# Autodesk Inventor assembly: ELEV_000_FULLASMBLY
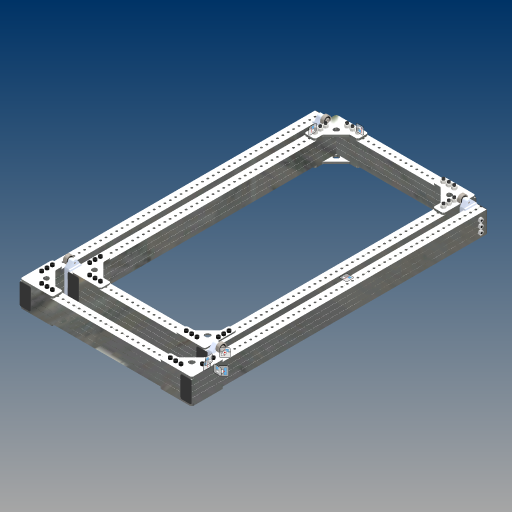
[picture p0: Inventor's stored thumbnail of the model, 512x512]
Saved by Autodesk Inventor 2024.3 (Build 283343000, 343)
## iProperties
Created: 2024-11-25
Part Number: ELEV_000_FULLASMBLY
Document SubType Name: Assembly
Designer: Kenji
Mass: 3407.89 g
Surface Area: 12378 cm^2
Volume: 1206.36 cm^3
Density: 2.82493 g/cm^3
Author: Kenji
## Documents named in this file (25)
- C:\Users\Kenji\Documents\GitHub\1622-2024-Casino-Clash-CAD-A-Thon\Elevator\ELEV_000_FULLASMBLY.iam
- C:\Users\Kenji\Documents\GitHub\1622-2024-Casino-Clash-CAD-A-Thon\Elevator\ELEV_001_BAR1(27.500 in).ipt
- C:\Users\Kenji\Documents\GitHub\1622-2024-Casino-Clash-CAD-A-Thon\Elevator\ELEV_002_BAR2(14.000 in).ipt
- C:\Users\Kenji\Documents\GitHub\1622-2024-Casino-Clash-CAD-A-Thon\Elevator\ELEV_003_BAR3(25.000 in).ipt
- C:\Users\Kenji\Documents\GitHub\1622-2024-Casino-Clash-CAD-A-Thon\COTS Library\Motion\BearingBlocks\ElevatorBlocks\WCP-0897_InlineBearingBlock.iam
- C:\Users\Kenji\Documents\GitHub\1622-2024-Casino-Clash-CAD-A-Thon\Elevator\ELEV_004_BAR4(12.000 in).ipt
- C:\Users\Kenji\Documents\GitHub\1622-2024-Casino-Clash-CAD-A-Thon\Elevator\ELEV_005_SUPBRK1.ipt
- C:\Users\Kenji\Documents\GitHub\1622-2024-Casino-Clash-CAD-A-Thon\COTS Library\Fasteners\Nuts\COTS_90633A411_Low-Strength Steel Thin Nylon-Insert Locknut_10-32.ipt
- C:\Users\Kenji\Documents\GitHub\1622-2024-Casino-Clash-CAD-A-Thon\Elevator\ELEV_006_SUPBRK1_THRD.ipt
- C:\Users\Kenji\Documents\GitHub\1622-2024-Casino-Clash-CAD-A-Thon\COTS Library\Fasteners\Bolts\Socket-Head\10-32\COTS_90044A121_Black-Oxide Alloy Steel Socket Head Screw_10-32_2.5in.ipt
- C:\Users\Kenji\Documents\GitHub\1622-2024-Casino-Clash-CAD-A-Thon\COTS Library\Fasteners\Bolts\Socket-Head\10-32\COTS_90044A202_Black-Oxide Alloy Steel Socket Head Screw_1-.375.ipt
- C:\Users\Kenji\Documents\GitHub\1622-2024-Casino-Clash-CAD-A-Thon\COTS Library\Fasteners\Bolts\Socket-Head\10-32\COTS_91251A342_Black-Oxide Alloy Steel Socket Head Screw_.5in.ipt
- C:\Users\Kenji\Documents\GitHub\1622-2024-Casino-Clash-CAD-A-Thon\Elevator\ELEV_007_SUPBRK2.ipt
- C:\Users\Kenji\Documents\GitHub\1622-2024-Casino-Clash-CAD-A-Thon\COTS Library\Fasteners\Bolts\Socket-Head\10-32\COTS_91251A359_Black-Oxide Alloy Steel Socket Head Screw_10-32_2_3-4in.ipt
- C:\Users\Kenji\Documents\GitHub\1622-2024-Casino-Clash-CAD-A-Thon\COTS Library\Fasteners\Nuts\COTS_90631A411_Low-Strength Steel Nylon-Insert Locknut_10-32.ipt
- C:\Users\Kenji\Documents\GitHub\1622-2024-Casino-Clash-CAD-A-Thon\Elevator\ELEV_008_SUPBRK3.ipt
- C:\Users\Kenji\Documents\GitHub\1622-2024-Casino-Clash-CAD-A-Thon\Elevator\ELEV_009_BOLTCOVER.ipt
- C:\Users\Kenji\Documents\GitHub\1622-2024-Casino-Clash-CAD-A-Thon\Elevator\ELEV_010_BOLTCOVER2.ipt
- C:\Users\Kenji\Documents\GitHub\1622-2024-Casino-Clash-CAD-A-Thon\Elevator\ELEV_011_EXTRUENDCAP.ipt
- C:\Users\Kenji\Documents\GitHub\1622-2024-Casino-Clash-CAD-A-Thon\Elevator\ELEV_000_FULLASMBLY\AIP\FEA\ew6g7bhkw.fins
- C:\Users\Kenji\Documents\GitHub\1622-2024-Casino-Clash-CAD-A-Thon\Elevator\ELEV_000_FULLASMBLY\AIP\FEA\ew6g7bhkw.fsat
- C:\Users\Kenji\Documents\GitHub\1622-2024-Casino-Clash-CAD-A-Thon\Elevator\ELEV_000_FULLASMBLY\AIP\FEA\ew6g7bhkw.ftes
- C:\Users\Kenji\Documents\GitHub\1622-2024-Casino-Clash-CAD-A-Thon\Elevator\ELEV_000_FULLASMBLY\AIP\FEA\ew6g7bhkw.fwiz
- C:\Users\Kenji\Documents\GitHub\1622-2024-Casino-Clash-CAD-A-Thon\Elevator\ELEV_000_FULLASMBLY\AIP\FEA\ew6g7biao.fmsh
- C:\Users\Kenji\Documents\GitHub\1622-2024-Casino-Clash-CAD-A-Thon\Elevator\ELEV_000_FULLASMBLY\AIP\FEA\ew6g7bibk.fres
## Components (151 placed, 18 different names)
1. ELEV_001_BAR1(27.500 in):1 — Flush:1, Flush:2, Mate:1, Mate:2, Flush:7, Tangent:2, Mate:10, Flush:11, Mate:11, Mate:78, Mate:133, Mate:136, Mate:137, Mate:181, Mate:183, Mate:184, Mate:201, Mate:202, Mate:203
2. ELEV_001_BAR1(27.500 in):2 — Flush:1, Flush:2, Mate:1, Flush:3, Flush:4, Mate:3, Angle:1, Mate:4, Flush:8, Angle:2, Mate:74, Mate:128, Mate:131, Mate:178, Mate:180, Mate:182, Mate:198, Mate:199, Mate:200
3. ELEV_002_BAR2(14.000 in):1 — Flush:3, Flush:4, Mate:2, Mate:127, Flush:24, Mate:132, Mate:134, Mate:135
4. ELEV_003_BAR3(25.000 in):1 — Flush:5, Flush:6, Flush:7, Mate:8, Flush:10, Mate:9, Mate:82, Flush:19, Flush:21, Mate:186, Mate:187, Mate:188, Mate:195, Mate:196, Mate:197
5. ELEV_003_BAR3(25.000 in):2 — Flush:5, Flush:6, Tangent:1, Angle:2, Mate:5, Angle:3, Mate:6, Flush:9, Mate:12, Flush:12, Flush:13, Mate:13, Flush:14, Mate:14, Mate:16, Mate:62, Mate:86, Flush:17, Flush:22, Mate:189, Mate:190, Mate:191, Mate:192, Mate:193, Mate:194
6. WCP-0897_InlineBearingBlock:1 [sub-assembly] — Mate:5, Angle:3, Mate:6, Flush:9, Mate:83, Mate:84
7. WCP-0897_InlineBearingBlock:2 [sub-assembly] — Mate:3, Angle:1, Mate:4, Tangent:1, Flush:8, Mate:71, Mate:72
8. WCP-0897_InlineBearingBlock:3 [sub-assembly] — Mate:8, Flush:10, Mate:9, Tangent:2, Mate:79, Mate:80
9. WCP-0897_InlineBearingBlock:4 [sub-assembly] — Mate:10, Flush:11, Mate:11, Mate:75, Mate:76
10. ELEV_004_BAR4(12.000 in):1 — Mate:12, Flush:12, Flush:13, Mate:17, Mate:18, Mate:19, Angle:4, Mate:20, Mate:42, Mate:45, Mate:60, Flush:15, Mate:61
11. ELEV_004_BAR4(12.000 in):2 — Mate:13, Flush:14, Mate:14, Flush:16, Flush:18, Mate:88, Flush:20, Mate:89, Flush:23, Mate:90, Mate:110
12. ELEV_005_SUPBRK1:1 — Mate:16, Mate:17, Mate:18, Mate:67, Mate:68, Mate:69, Mate:70
13. ELEV_005_SUPBRK1:2 — Mate:19, Angle:4, Mate:20, Mate:63, Mate:64, Mate:65, Mate:66
14. ELEV_006_SUPBRK1_THRD:1 — Mate:42, Mate:61, Mate:62, Mate:159, Mate:161
15. ELEV_006_SUPBRK1_THRD:2 — Mate:45, Mate:60, Flush:15, Mate:155, Mate:157
16. ELEV_007_SUPBRK2:1 — Flush:16, Flush:17, Mate:110, Mate:120, Mate:122
17. ELEV_007_SUPBRK2:2 — Flush:18, Flush:19, Mate:88, Mate:124, Mate:126
18. ELEV_007_SUPBRK2:3 — Flush:22, Flush:23, Mate:90, Mate:115, Mate:116, Mate:117, Mate:118
19. ELEV_007_SUPBRK2:4 — Flush:20, Flush:21, Mate:89, Mate:111, Mate:112, Mate:113, Mate:114
20. ELEV_008_SUPBRK3:1 — Mate:127, Flush:24, Mate:128, Mate:129, Mate:130, Mate:138, Mate:139, Mate:144, Mate:145
21. ELEV_008_SUPBRK3:2 — Mate:129, Mate:130, Mate:131, Mate:148, Mate:149
22. ELEV_008_SUPBRK3:3 — Mate:132, Mate:133, Mate:134, Mate:151, Mate:153
23. ELEV_008_SUPBRK3:4 — Mate:135, Mate:136, Mate:137, Mate:140, Mate:141, Mate:142, Mate:143
24. ELEV_011_EXTRUENDCAP:1 — Mate:189, Mate:190, Mate:191
25. ELEV_011_EXTRUENDCAP:2 — Mate:178, Mate:180, Mate:182
26. ELEV_011_EXTRUENDCAP:3 — Mate:186, Mate:187, Mate:188
27. ELEV_011_EXTRUENDCAP:4 — Mate:181, Mate:183, Mate:184
28. ELEV_011_EXTRUENDCAP:5 — Mate:198, Mate:199, Mate:200
29. ELEV_011_EXTRUENDCAP:6 — Mate:201, Mate:202, Mate:203
30. ELEV_011_EXTRUENDCAP:7 — Mate:192, Mate:193, Mate:194
31. ELEV_011_EXTRUENDCAP:8 — Mate:195, Mate:196, Mate:197
32. COTS_90044A121_Black-Oxide Alloy Steel Socket Head Screw_10-32_2.5in:1 — Mate:63, Mate:64
33. COTS_90044A121_Black-Oxide Alloy Steel Socket Head Screw_10-32_2.5in:5
34. COTS_90044A121_Black-Oxide Alloy Steel Socket Head Screw_10-32_2.5in:6 — Mate:156
35. COTS_90044A121_Black-Oxide Alloy Steel Socket Head Screw_10-32_2.5in:4 — Mate:65, Mate:66
36. COTS_90044A121_Black-Oxide Alloy Steel Socket Head Screw_10-32_2.5in:7
37. COTS_90044A121_Black-Oxide Alloy Steel Socket Head Screw_10-32_2.5in:8 — Mate:154
38. COTS_90044A121_Black-Oxide Alloy Steel Socket Head Screw_10-32_2.5in:3 — Mate:68, Mate:70
39. COTS_90044A121_Black-Oxide Alloy Steel Socket Head Screw_10-32_2.5in:9
40. COTS_90044A121_Black-Oxide Alloy Steel Socket Head Screw_10-32_2.5in:10 — Mate:160
41. COTS_90044A121_Black-Oxide Alloy Steel Socket Head Screw_10-32_2.5in:2 — Mate:67, Mate:69
42. COTS_90044A121_Black-Oxide Alloy Steel Socket Head Screw_10-32_2.5in:11
43. COTS_90044A121_Black-Oxide Alloy Steel Socket Head Screw_10-32_2.5in:12 — Mate:158
44. COTS_90044A202_Black-Oxide Alloy Steel Socket Head Screw_1-.375:1 — Mate:71, Mate:72, Mate:73
45. COTS_90633A411_Low-Strength Steel Thin Nylon-Insert Locknut_10-32:1 — Mate:73, Mate:74
46. COTS_90044A202_Black-Oxide Alloy Steel Socket Head Screw_1-.375:2
47. COTS_90633A411_Low-Strength Steel Thin Nylon-Insert Locknut_10-32:2
48. COTS_90044A202_Black-Oxide Alloy Steel Socket Head Screw_1-.375:3
49. COTS_90633A411_Low-Strength Steel Thin Nylon-Insert Locknut_10-32:3
50. COTS_90633A411_Low-Strength Steel Thin Nylon-Insert Locknut_10-32:4 — Mate:77, Mate:78
51. COTS_90044A202_Black-Oxide Alloy Steel Socket Head Screw_1-.375:4 — Mate:75, Mate:76, Mate:77
52. COTS_90633A411_Low-Strength Steel Thin Nylon-Insert Locknut_10-32:5
53. COTS_90044A202_Black-Oxide Alloy Steel Socket Head Screw_1-.375:5
54. COTS_90633A411_Low-Strength Steel Thin Nylon-Insert Locknut_10-32:6
55. COTS_90044A202_Black-Oxide Alloy Steel Socket Head Screw_1-.375:6
56. COTS_91251A342_Black-Oxide Alloy Steel Socket Head Screw_.5in:1 — Mate:79, Mate:80, Mate:81
57. COTS_90633A411_Low-Strength Steel Thin Nylon-Insert Locknut_10-32:7 — Mate:81, Mate:82
58. COTS_91251A342_Black-Oxide Alloy Steel Socket Head Screw_.5in:2
59. COTS_90633A411_Low-Strength Steel Thin Nylon-Insert Locknut_10-32:8
60. COTS_91251A342_Black-Oxide Alloy Steel Socket Head Screw_.5in:3
61. COTS_90633A411_Low-Strength Steel Thin Nylon-Insert Locknut_10-32:9
62. COTS_90633A411_Low-Strength Steel Thin Nylon-Insert Locknut_10-32:10 — Mate:85, Mate:86
63. COTS_91251A342_Black-Oxide Alloy Steel Socket Head Screw_.5in:4 — Mate:83, Mate:84, Mate:85
64. COTS_90633A411_Low-Strength Steel Thin Nylon-Insert Locknut_10-32:11
65. COTS_91251A342_Black-Oxide Alloy Steel Socket Head Screw_.5in:5
66. COTS_90633A411_Low-Strength Steel Thin Nylon-Insert Locknut_10-32:12
67. COTS_91251A342_Black-Oxide Alloy Steel Socket Head Screw_.5in:6
68. COTS_91251A359_Black-Oxide Alloy Steel Socket Head Screw_10-32_2_3-4in:3 — Mate:111, Mate:112, Mate:123, Mate:166
69. COTS_90631A411_Low-Strength Steel Nylon-Insert Locknut_10-32:2 — Mate:123, Mate:124, Mate:168
70. COTS_91251A359_Black-Oxide Alloy Steel Socket Head Screw_10-32_2_3-4in:5
71. COTS_90631A411_Low-Strength Steel Nylon-Insert Locknut_10-32:5
72. COTS_91251A359_Black-Oxide Alloy Steel Socket Head Screw_10-32_2_3-4in:6
73. COTS_90631A411_Low-Strength Steel Nylon-Insert Locknut_10-32:6
74. COTS_91251A359_Black-Oxide Alloy Steel Socket Head Screw_10-32_2_3-4in:1 — Mate:113, Mate:114, Mate:125, Mate:167
75. COTS_91251A359_Black-Oxide Alloy Steel Socket Head Screw_10-32_2_3-4in:7
76. COTS_91251A359_Black-Oxide Alloy Steel Socket Head Screw_10-32_2_3-4in:8
77. COTS_91251A359_Black-Oxide Alloy Steel Socket Head Screw_10-32_2_3-4in:2 — Mate:115, Mate:118, Mate:121, Mate:163
78. COTS_90631A411_Low-Strength Steel Nylon-Insert Locknut_10-32:4 — Mate:121, Mate:122, Mate:164
79. COTS_91251A359_Black-Oxide Alloy Steel Socket Head Screw_10-32_2_3-4in:9
80. COTS_90631A411_Low-Strength Steel Nylon-Insert Locknut_10-32:7
81. COTS_91251A359_Black-Oxide Alloy Steel Socket Head Screw_10-32_2_3-4in:10
82. COTS_90631A411_Low-Strength Steel Nylon-Insert Locknut_10-32:8
83. COTS_90631A411_Low-Strength Steel Nylon-Insert Locknut_10-32:3 — Mate:119, Mate:120, Mate:165
84. COTS_91251A359_Black-Oxide Alloy Steel Socket Head Screw_10-32_2_3-4in:4 — Mate:116, Mate:117, Mate:119, Mate:162
85. COTS_90631A411_Low-Strength Steel Nylon-Insert Locknut_10-32:9
86. COTS_91251A359_Black-Oxide Alloy Steel Socket Head Screw_10-32_2_3-4in:11
87. COTS_90631A411_Low-Strength Steel Nylon-Insert Locknut_10-32:10
88. COTS_91251A359_Black-Oxide Alloy Steel Socket Head Screw_10-32_2_3-4in:12
89. COTS_90631A411_Low-Strength Steel Nylon-Insert Locknut_10-32:1 — Mate:125, Mate:126, Mate:169
90. COTS_90631A411_Low-Strength Steel Nylon-Insert Locknut_10-32:11
91. COTS_90631A411_Low-Strength Steel Nylon-Insert Locknut_10-32:12
92. COTS_90631A411_Low-Strength Steel Nylon-Insert Locknut_10-32:14 — Mate:152, Mate:153, Mate:172
93. COTS_91251A359_Black-Oxide Alloy Steel Socket Head Screw_10-32_2_3-4in:14 — Mate:140, Mate:143, Mate:152, Mate:171
94. COTS_90631A411_Low-Strength Steel Nylon-Insert Locknut_10-32:17
95. COTS_91251A359_Black-Oxide Alloy Steel Socket Head Screw_10-32_2_3-4in:17
96. COTS_90631A411_Low-Strength Steel Nylon-Insert Locknut_10-32:18
97. COTS_91251A359_Black-Oxide Alloy Steel Socket Head Screw_10-32_2_3-4in:18
98. COTS_91251A359_Black-Oxide Alloy Steel Socket Head Screw_10-32_2_3-4in:13 — Mate:141, Mate:142, Mate:150, Mate:170
99. COTS_90631A411_Low-Strength Steel Nylon-Insert Locknut_10-32:15 — Mate:150, Mate:151, Mate:173
100. COTS_91251A359_Black-Oxide Alloy Steel Socket Head Screw_10-32_2_3-4in:19
101. COTS_90631A411_Low-Strength Steel Nylon-Insert Locknut_10-32:19
102. COTS_91251A359_Black-Oxide Alloy Steel Socket Head Screw_10-32_2_3-4in:20
103. COTS_90631A411_Low-Strength Steel Nylon-Insert Locknut_10-32:20
104. COTS_91251A359_Black-Oxide Alloy Steel Socket Head Screw_10-32_2_3-4in:15 — Mate:139, Mate:145, Mate:147, Mate:174
105. COTS_90631A411_Low-Strength Steel Nylon-Insert Locknut_10-32:13 — Mate:147, Mate:149, Mate:175
106. COTS_91251A359_Black-Oxide Alloy Steel Socket Head Screw_10-32_2_3-4in:21
107. COTS_90631A411_Low-Strength Steel Nylon-Insert Locknut_10-32:21
108. COTS_91251A359_Black-Oxide Alloy Steel Socket Head Screw_10-32_2_3-4in:22
109. COTS_90631A411_Low-Strength Steel Nylon-Insert Locknut_10-32:22
110. COTS_90631A411_Low-Strength Steel Nylon-Insert Locknut_10-32:16 — Mate:146, Mate:148, Mate:177
111. COTS_91251A359_Black-Oxide Alloy Steel Socket Head Screw_10-32_2_3-4in:16 — Mate:138, Mate:144, Mate:146, Mate:176
112. COTS_90631A411_Low-Strength Steel Nylon-Insert Locknut_10-32:23
113. COTS_91251A359_Black-Oxide Alloy Steel Socket Head Screw_10-32_2_3-4in:23
114. COTS_90631A411_Low-Strength Steel Nylon-Insert Locknut_10-32:24
115. COTS_91251A359_Black-Oxide Alloy Steel Socket Head Screw_10-32_2_3-4in:24
116. ELEV_009_BOLTCOVER:2 — Mate:156, Mate:157
117. ELEV_009_BOLTCOVER:5
118. ELEV_009_BOLTCOVER:6
119. ELEV_009_BOLTCOVER:1 — Mate:154, Mate:155
120. ELEV_009_BOLTCOVER:7
121. ELEV_009_BOLTCOVER:8
122. ELEV_009_BOLTCOVER:3 — Mate:160, Mate:161
123. ELEV_009_BOLTCOVER:9
124. ELEV_009_BOLTCOVER:10
125. ELEV_009_BOLTCOVER:4 — Mate:158, Mate:159
126. ELEV_009_BOLTCOVER:11
127. ELEV_009_BOLTCOVER:12
128. ELEV_010_BOLTCOVER2:2 — Mate:163, Mate:164
129. ELEV_010_BOLTCOVER2:5
130. ELEV_010_BOLTCOVER2:6
131. ELEV_010_BOLTCOVER2:1 — Mate:162, Mate:165
132. ELEV_010_BOLTCOVER2:7
133. ELEV_010_BOLTCOVER2:8
134. ELEV_010_BOLTCOVER2:3 — Mate:167, Mate:169
135. ELEV_010_BOLTCOVER2:9
136. ELEV_010_BOLTCOVER2:10
137. ELEV_010_BOLTCOVER2:4 — Mate:166, Mate:168
138. ELEV_010_BOLTCOVER2:11
139. ELEV_010_BOLTCOVER2:12
140. ELEV_010_BOLTCOVER2:16 — Mate:170, Mate:173
141. ELEV_010_BOLTCOVER2:17
142. ELEV_010_BOLTCOVER2:18
143. ELEV_010_BOLTCOVER2:15 — Mate:171, Mate:172
144. ELEV_010_BOLTCOVER2:19
145. ELEV_010_BOLTCOVER2:20
146. ELEV_010_BOLTCOVER2:14 — Mate:174, Mate:175
147. ELEV_010_BOLTCOVER2:21
148. ELEV_010_BOLTCOVER2:22
149. ELEV_010_BOLTCOVER2:13 — Mate:176, Mate:177
150. ELEV_010_BOLTCOVER2:23
151. ELEV_010_BOLTCOVER2:24
## Component patterns: (3 elements, first: COTS_90044A121_Black-Oxide Alloy Steel Socket Head Screw_10-32_2.5in:1), (3 elements, first: COTS_90044A121_Black-Oxide Alloy Steel Socket Head Screw_10-32_2.5in:4), (3 elements, first: COTS_90044A121_Black-Oxide Alloy Steel Socket Head Screw_10-32_2.5in:3), (3 elements, first: COTS_90044A121_Black-Oxide Alloy Steel Socket Head Screw_10-32_2.5in:2), (3 elements, first: COTS_90044A202_Black-Oxide Alloy Steel Socket Head Screw_1-.375:1 + COTS_90633A411_Low-Strength Steel Thin Nylon-Insert Locknut_10-32:1), (3 elements, first: COTS_90633A411_Low-Strength Steel Thin Nylon-Insert Locknut_10-32:4 + COTS_90044A202_Black-Oxide Alloy Steel Socket Head Screw_1-.375:4), (3 elements, first: COTS_91251A342_Black-Oxide Alloy Steel Socket Head Screw_.5in:1 + COTS_90633A411_Low-Strength Steel Thin Nylon-Insert Locknut_10-32:7), (3 elements, first: COTS_90633A411_Low-Strength Steel Thin Nylon-Insert Locknut_10-32:10 + COTS_91251A342_Black-Oxide Alloy Steel Socket Head Screw_.5in:4), (3 elements, first: COTS_91251A359_Black-Oxide Alloy Steel Socket Head Screw_10-32_2_3-4in:3 + COTS_90631A411_Low-Strength Steel Nylon-Insert Locknut_10-32:2), (3 elements, first: COTS_91251A359_Black-Oxide Alloy Steel Socket Head Screw_10-32_2_3-4in:1), (3 elements, first: COTS_91251A359_Black-Oxide Alloy Steel Socket Head Screw_10-32_2_3-4in:2 + COTS_90631A411_Low-Strength Steel Nylon-Insert Locknut_10-32:4), (3 elements, first: COTS_90631A411_Low-Strength Steel Nylon-Insert Locknut_10-32:3 + COTS_91251A359_Black-Oxide Alloy Steel Socket Head Screw_10-32_2_3-4in:4), (3 elements, first: COTS_90631A411_Low-Strength Steel Nylon-Insert Locknut_10-32:1), (3 elements, first: COTS_90631A411_Low-Strength Steel Nylon-Insert Locknut_10-32:14 + COTS_91251A359_Black-Oxide Alloy Steel Socket Head Screw_10-32_2_3-4in:14), (3 elements, first: COTS_91251A359_Black-Oxide Alloy Steel Socket Head Screw_10-32_2_3-4in:13 + COTS_90631A411_Low-Strength Steel Nylon-Insert Locknut_10-32:15), (3 elements, first: COTS_91251A359_Black-Oxide Alloy Steel Socket Head Screw_10-32_2_3-4in:15 + COTS_90631A411_Low-Strength Steel Nylon-Insert Locknut_10-32:13), (3 elements, first: COTS_90631A411_Low-Strength Steel Nylon-Insert Locknut_10-32:16 + COTS_91251A359_Black-Oxide Alloy Steel Socket Head Screw_10-32_2_3-4in:16), (3 elements, first: ELEV_009_BOLTCOVER:2), (3 elements, first: ELEV_009_BOLTCOVER:1), (3 elements, first: ELEV_009_BOLTCOVER:3), (3 elements, first: ELEV_009_BOLTCOVER:4), (3 elements, first: ELEV_010_BOLTCOVER2:2), (3 elements, first: ELEV_010_BOLTCOVER2:1), (3 elements, first: ELEV_010_BOLTCOVER2:3), (3 elements, first: ELEV_010_BOLTCOVER2:4), (3 elements, first: ELEV_010_BOLTCOVER2:16), (3 elements, first: ELEV_010_BOLTCOVER2:15), (3 elements, first: ELEV_010_BOLTCOVER2:14), (3 elements, first: ELEV_010_BOLTCOVER2:13)
## Relationships (172: Mate 142, Flush 24, Angle 4, Tangent 2)
- Flush:1: ELEV_001_BAR1(27.500 in):1 ↔ ELEV_001_BAR1(27.500 in):2
- Flush:2: ELEV_001_BAR1(27.500 in):1 ↔ ELEV_001_BAR1(27.500 in):2
- Mate:1 (355.6 mm): ELEV_001_BAR1(27.500 in):1 ↔ ELEV_001_BAR1(27.500 in):2
- Flush:3: ELEV_001_BAR1(27.500 in):2 ↔ ELEV_002_BAR2(14.000 in):1
- Flush:4: ELEV_001_BAR1(27.500 in):2 ↔ ELEV_002_BAR2(14.000 in):1
- Mate:2: ELEV_001_BAR1(27.500 in):1 ↔ ELEV_002_BAR2(14.000 in):1
- Flush:5: ELEV_003_BAR3(25.000 in):1 ↔ ELEV_003_BAR3(25.000 in):2
- Flush:6: ELEV_003_BAR3(25.000 in):1 ↔ ELEV_003_BAR3(25.000 in):2
- Flush:7: ELEV_001_BAR1(27.500 in):1 ↔ ELEV_003_BAR3(25.000 in):1
- Mate:3: ELEV_001_BAR1(27.500 in):2 ↔ WCP-0897_InlineBearingBlock:2
- Angle:1 (0 deg): ELEV_001_BAR1(27.500 in):2 ↔ WCP-0897_InlineBearingBlock:2
- Mate:4: ELEV_001_BAR1(27.500 in):2 ↔ WCP-0897_InlineBearingBlock:2
- Tangent:1: ELEV_003_BAR3(25.000 in):2 ↔ WCP-0897_InlineBearingBlock:2
- Flush:8: ELEV_001_BAR1(27.500 in):2 ↔ WCP-0897_InlineBearingBlock:2
- Angle:2 (0 deg): ELEV_001_BAR1(27.500 in):2 ↔ ELEV_003_BAR3(25.000 in):2
- Mate:5: ELEV_003_BAR3(25.000 in):2 ↔ WCP-0897_InlineBearingBlock:1
- Angle:3 (0 deg): ELEV_003_BAR3(25.000 in):2 ↔ WCP-0897_InlineBearingBlock:1
- Mate:6: ELEV_003_BAR3(25.000 in):2 ↔ WCP-0897_InlineBearingBlock:1
- Flush:9: ELEV_003_BAR3(25.000 in):2 ↔ WCP-0897_InlineBearingBlock:1
- Mate:8: ELEV_003_BAR3(25.000 in):1 ↔ WCP-0897_InlineBearingBlock:3
- Flush:10: ELEV_003_BAR3(25.000 in):1 ↔ WCP-0897_InlineBearingBlock:3
- Mate:9: ELEV_003_BAR3(25.000 in):1 ↔ WCP-0897_InlineBearingBlock:3
- Tangent:2: ELEV_001_BAR1(27.500 in):1 ↔ WCP-0897_InlineBearingBlock:3
- Mate:10: ELEV_001_BAR1(27.500 in):1 ↔ WCP-0897_InlineBearingBlock:4
- Flush:11: ELEV_001_BAR1(27.500 in):1 ↔ WCP-0897_InlineBearingBlock:4
- Mate:11: ELEV_001_BAR1(27.500 in):1 ↔ WCP-0897_InlineBearingBlock:4
- Mate:12: ELEV_003_BAR3(25.000 in):2 ↔ ELEV_004_BAR4(12.000 in):1
- Flush:12: ELEV_003_BAR3(25.000 in):2 ↔ ELEV_004_BAR4(12.000 in):1
- Flush:13: ELEV_003_BAR3(25.000 in):2 ↔ ELEV_004_BAR4(12.000 in):1
- Mate:13: ELEV_003_BAR3(25.000 in):2 ↔ ELEV_004_BAR4(12.000 in):2
- Flush:14: ELEV_003_BAR3(25.000 in):2 ↔ ELEV_004_BAR4(12.000 in):2
- Mate:14: ELEV_003_BAR3(25.000 in):2 ↔ ELEV_004_BAR4(12.000 in):2
- Mate:16: ELEV_003_BAR3(25.000 in):2 ↔ ELEV_005_SUPBRK1:1
- Mate:17: ELEV_004_BAR4(12.000 in):1 ↔ ELEV_005_SUPBRK1:1
- Mate:18: ELEV_004_BAR4(12.000 in):1 ↔ ELEV_005_SUPBRK1:1
- Mate:19: ELEV_004_BAR4(12.000 in):1 ↔ ELEV_005_SUPBRK1:2
- Angle:4 (0 deg): ELEV_004_BAR4(12.000 in):1 ↔ ELEV_005_SUPBRK1:2
- Mate:20: ELEV_004_BAR4(12.000 in):1 ↔ ELEV_005_SUPBRK1:2
- Mate:42: ELEV_004_BAR4(12.000 in):1 ↔ ELEV_006_SUPBRK1_THRD:1
- Mate:45: ELEV_004_BAR4(12.000 in):1 ↔ ELEV_006_SUPBRK1_THRD:2
- Mate:60: ELEV_004_BAR4(12.000 in):1 ↔ ELEV_006_SUPBRK1_THRD:2
- Flush:15: ELEV_004_BAR4(12.000 in):1 ↔ ELEV_006_SUPBRK1_THRD:2
- Mate:61: ELEV_004_BAR4(12.000 in):1 ↔ ELEV_006_SUPBRK1_THRD:1
- Mate:62: ELEV_003_BAR3(25.000 in):2 ↔ ELEV_006_SUPBRK1_THRD:1
- Mate:63: ELEV_005_SUPBRK1:2 ↔ COTS_90044A121_Black-Oxide Alloy Steel Socket Head Screw_10-32_2.5in:1
- Mate:64: ELEV_005_SUPBRK1:2 ↔ COTS_90044A121_Black-Oxide Alloy Steel Socket Head Screw_10-32_2.5in:1
- Mate:65: ELEV_005_SUPBRK1:2 ↔ COTS_90044A121_Black-Oxide Alloy Steel Socket Head Screw_10-32_2.5in:4
- Mate:66: ELEV_005_SUPBRK1:2 ↔ COTS_90044A121_Black-Oxide Alloy Steel Socket Head Screw_10-32_2.5in:4
- Mate:67: ELEV_005_SUPBRK1:1 ↔ COTS_90044A121_Black-Oxide Alloy Steel Socket Head Screw_10-32_2.5in:2
- Mate:68: ELEV_005_SUPBRK1:1 ↔ COTS_90044A121_Black-Oxide Alloy Steel Socket Head Screw_10-32_2.5in:3
- Mate:69: ELEV_005_SUPBRK1:1 ↔ COTS_90044A121_Black-Oxide Alloy Steel Socket Head Screw_10-32_2.5in:2
- Mate:70: ELEV_005_SUPBRK1:1 ↔ COTS_90044A121_Black-Oxide Alloy Steel Socket Head Screw_10-32_2.5in:3
- Mate:71: WCP-0897_InlineBearingBlock:2 ↔ COTS_90044A202_Black-Oxide Alloy Steel Socket Head Screw_1-.375:1
- Mate:72: WCP-0897_InlineBearingBlock:2 ↔ COTS_90044A202_Black-Oxide Alloy Steel Socket Head Screw_1-.375:1
- Mate:73: COTS_90044A202_Black-Oxide Alloy Steel Socket Head Screw_1-.375:1 ↔ COTS_90633A411_Low-Strength Steel Thin Nylon-Insert Locknut_10-32:1
- Mate:74: ELEV_001_BAR1(27.500 in):2 ↔ COTS_90633A411_Low-Strength Steel Thin Nylon-Insert Locknut_10-32:1
- Mate:75: WCP-0897_InlineBearingBlock:4 ↔ COTS_90044A202_Black-Oxide Alloy Steel Socket Head Screw_1-.375:4
- Mate:76: WCP-0897_InlineBearingBlock:4 ↔ COTS_90044A202_Black-Oxide Alloy Steel Socket Head Screw_1-.375:4
- Mate:77: COTS_90633A411_Low-Strength Steel Thin Nylon-Insert Locknut_10-32:4 ↔ COTS_90044A202_Black-Oxide Alloy Steel Socket Head Screw_1-.375:4
- Mate:78: ELEV_001_BAR1(27.500 in):1 ↔ COTS_90633A411_Low-Strength Steel Thin Nylon-Insert Locknut_10-32:4
- Mate:79: WCP-0897_InlineBearingBlock:3 ↔ COTS_91251A342_Black-Oxide Alloy Steel Socket Head Screw_.5in:1
- Mate:80: WCP-0897_InlineBearingBlock:3 ↔ COTS_91251A342_Black-Oxide Alloy Steel Socket Head Screw_.5in:1
- Mate:81: COTS_91251A342_Black-Oxide Alloy Steel Socket Head Screw_.5in:1 ↔ COTS_90633A411_Low-Strength Steel Thin Nylon-Insert Locknut_10-32:7
- Mate:82: ELEV_003_BAR3(25.000 in):1 ↔ COTS_90633A411_Low-Strength Steel Thin Nylon-Insert Locknut_10-32:7
- Mate:83: WCP-0897_InlineBearingBlock:1 ↔ COTS_91251A342_Black-Oxide Alloy Steel Socket Head Screw_.5in:4
- Mate:84: WCP-0897_InlineBearingBlock:1 ↔ COTS_91251A342_Black-Oxide Alloy Steel Socket Head Screw_.5in:4
- Mate:85: COTS_90633A411_Low-Strength Steel Thin Nylon-Insert Locknut_10-32:10 ↔ COTS_91251A342_Black-Oxide Alloy Steel Socket Head Screw_.5in:4
- Mate:86: ELEV_003_BAR3(25.000 in):2 ↔ COTS_90633A411_Low-Strength Steel Thin Nylon-Insert Locknut_10-32:10
- Flush:16: ELEV_004_BAR4(12.000 in):2 ↔ ELEV_007_SUPBRK2:1
- Flush:17: ELEV_003_BAR3(25.000 in):2 ↔ ELEV_007_SUPBRK2:1
- Flush:18: ELEV_004_BAR4(12.000 in):2 ↔ ELEV_007_SUPBRK2:2
- Flush:19: ELEV_003_BAR3(25.000 in):1 ↔ ELEV_007_SUPBRK2:2
- Mate:88: ELEV_004_BAR4(12.000 in):2 ↔ ELEV_007_SUPBRK2:2
- Flush:20: ELEV_004_BAR4(12.000 in):2 ↔ ELEV_007_SUPBRK2:4
- Flush:21: ELEV_003_BAR3(25.000 in):1 ↔ ELEV_007_SUPBRK2:4
- Mate:89: ELEV_004_BAR4(12.000 in):2 ↔ ELEV_007_SUPBRK2:4
- Flush:22: ELEV_003_BAR3(25.000 in):2 ↔ ELEV_007_SUPBRK2:3
- Flush:23: ELEV_004_BAR4(12.000 in):2 ↔ ELEV_007_SUPBRK2:3
- Mate:90: ELEV_004_BAR4(12.000 in):2 ↔ ELEV_007_SUPBRK2:3
- Mate:110: ELEV_004_BAR4(12.000 in):2 ↔ ELEV_007_SUPBRK2:1
- Mate:111: ELEV_007_SUPBRK2:4 ↔ COTS_91251A359_Black-Oxide Alloy Steel Socket Head Screw_10-32_2_3-4in:3
- Mate:112: ELEV_007_SUPBRK2:4 ↔ COTS_91251A359_Black-Oxide Alloy Steel Socket Head Screw_10-32_2_3-4in:3
- Mate:113: ELEV_007_SUPBRK2:4 ↔ COTS_91251A359_Black-Oxide Alloy Steel Socket Head Screw_10-32_2_3-4in:1
- Mate:114: ELEV_007_SUPBRK2:4 ↔ COTS_91251A359_Black-Oxide Alloy Steel Socket Head Screw_10-32_2_3-4in:1
- Mate:115: ELEV_007_SUPBRK2:3 ↔ COTS_91251A359_Black-Oxide Alloy Steel Socket Head Screw_10-32_2_3-4in:2
- Mate:116: ELEV_007_SUPBRK2:3 ↔ COTS_91251A359_Black-Oxide Alloy Steel Socket Head Screw_10-32_2_3-4in:4
- Mate:117: ELEV_007_SUPBRK2:3 ↔ COTS_91251A359_Black-Oxide Alloy Steel Socket Head Screw_10-32_2_3-4in:4
- Mate:118: ELEV_007_SUPBRK2:3 ↔ COTS_91251A359_Black-Oxide Alloy Steel Socket Head Screw_10-32_2_3-4in:2
- Mate:119: COTS_90631A411_Low-Strength Steel Nylon-Insert Locknut_10-32:3 ↔ COTS_91251A359_Black-Oxide Alloy Steel Socket Head Screw_10-32_2_3-4in:4
- Mate:120: ELEV_007_SUPBRK2:1 ↔ COTS_90631A411_Low-Strength Steel Nylon-Insert Locknut_10-32:3
- Mate:121: COTS_91251A359_Black-Oxide Alloy Steel Socket Head Screw_10-32_2_3-4in:2 ↔ COTS_90631A411_Low-Strength Steel Nylon-Insert Locknut_10-32:4
- Mate:122: ELEV_007_SUPBRK2:1 ↔ COTS_90631A411_Low-Strength Steel Nylon-Insert Locknut_10-32:4
- Mate:123: COTS_91251A359_Black-Oxide Alloy Steel Socket Head Screw_10-32_2_3-4in:3 ↔ COTS_90631A411_Low-Strength Steel Nylon-Insert Locknut_10-32:2
- Mate:124: ELEV_007_SUPBRK2:2 ↔ COTS_90631A411_Low-Strength Steel Nylon-Insert Locknut_10-32:2
- Mate:125: COTS_91251A359_Black-Oxide Alloy Steel Socket Head Screw_10-32_2_3-4in:1 ↔ COTS_90631A411_Low-Strength Steel Nylon-Insert Locknut_10-32:1
- Mate:126: ELEV_007_SUPBRK2:2 ↔ COTS_90631A411_Low-Strength Steel Nylon-Insert Locknut_10-32:1
- Mate:127: ELEV_002_BAR2(14.000 in):1 ↔ ELEV_008_SUPBRK3:1
- Flush:24: ELEV_002_BAR2(14.000 in):1 ↔ ELEV_008_SUPBRK3:1
- Mate:128: ELEV_001_BAR1(27.500 in):2 ↔ ELEV_008_SUPBRK3:1
- Mate:129: ELEV_008_SUPBRK3:1 ↔ ELEV_008_SUPBRK3:2
- Mate:130: ELEV_008_SUPBRK3:1 ↔ ELEV_008_SUPBRK3:2
- Mate:131: ELEV_001_BAR1(27.500 in):2 ↔ ELEV_008_SUPBRK3:2
- Mate:132: ELEV_002_BAR2(14.000 in):1 ↔ ELEV_008_SUPBRK3:3
- Mate:133: ELEV_001_BAR1(27.500 in):1 ↔ ELEV_008_SUPBRK3:3
- Mate:134: ELEV_002_BAR2(14.000 in):1 ↔ ELEV_008_SUPBRK3:3
- Mate:135: ELEV_002_BAR2(14.000 in):1 ↔ ELEV_008_SUPBRK3:4
- Mate:136: ELEV_001_BAR1(27.500 in):1 ↔ ELEV_008_SUPBRK3:4
- Mate:137: ELEV_001_BAR1(27.500 in):1 ↔ ELEV_008_SUPBRK3:4
- Mate:138: ELEV_008_SUPBRK3:1 ↔ COTS_91251A359_Black-Oxide Alloy Steel Socket Head Screw_10-32_2_3-4in:16
- Mate:139: ELEV_008_SUPBRK3:1 ↔ COTS_91251A359_Black-Oxide Alloy Steel Socket Head Screw_10-32_2_3-4in:15
- Mate:140: ELEV_008_SUPBRK3:4 ↔ COTS_91251A359_Black-Oxide Alloy Steel Socket Head Screw_10-32_2_3-4in:14
- Mate:141: ELEV_008_SUPBRK3:4 ↔ COTS_91251A359_Black-Oxide Alloy Steel Socket Head Screw_10-32_2_3-4in:13
- Mate:142: ELEV_008_SUPBRK3:4 ↔ COTS_91251A359_Black-Oxide Alloy Steel Socket Head Screw_10-32_2_3-4in:13
- Mate:143: ELEV_008_SUPBRK3:4 ↔ COTS_91251A359_Black-Oxide Alloy Steel Socket Head Screw_10-32_2_3-4in:14
- Mate:144: ELEV_008_SUPBRK3:1 ↔ COTS_91251A359_Black-Oxide Alloy Steel Socket Head Screw_10-32_2_3-4in:16
- Mate:145: ELEV_008_SUPBRK3:1 ↔ COTS_91251A359_Black-Oxide Alloy Steel Socket Head Screw_10-32_2_3-4in:15
- Mate:146: COTS_90631A411_Low-Strength Steel Nylon-Insert Locknut_10-32:16 ↔ COTS_91251A359_Black-Oxide Alloy Steel Socket Head Screw_10-32_2_3-4in:16
- Mate:147: COTS_91251A359_Black-Oxide Alloy Steel Socket Head Screw_10-32_2_3-4in:15 ↔ COTS_90631A411_Low-Strength Steel Nylon-Insert Locknut_10-32:13
- Mate:148: ELEV_008_SUPBRK3:2 ↔ COTS_90631A411_Low-Strength Steel Nylon-Insert Locknut_10-32:16
- Mate:149: ELEV_008_SUPBRK3:2 ↔ COTS_90631A411_Low-Strength Steel Nylon-Insert Locknut_10-32:13
- Mate:150: COTS_91251A359_Black-Oxide Alloy Steel Socket Head Screw_10-32_2_3-4in:13 ↔ COTS_90631A411_Low-Strength Steel Nylon-Insert Locknut_10-32:15
- Mate:151: ELEV_008_SUPBRK3:3 ↔ COTS_90631A411_Low-Strength Steel Nylon-Insert Locknut_10-32:15
- Mate:152: COTS_90631A411_Low-Strength Steel Nylon-Insert Locknut_10-32:14 ↔ COTS_91251A359_Black-Oxide Alloy Steel Socket Head Screw_10-32_2_3-4in:14
- Mate:153: ELEV_008_SUPBRK3:3 ↔ COTS_90631A411_Low-Strength Steel Nylon-Insert Locknut_10-32:14
- Mate:154: COTS_90044A121_Black-Oxide Alloy Steel Socket Head Screw_10-32_2.5in:8 ↔ ELEV_009_BOLTCOVER:1
- Mate:155: ELEV_006_SUPBRK1_THRD:2 ↔ ELEV_009_BOLTCOVER:1
- Mate:156: COTS_90044A121_Black-Oxide Alloy Steel Socket Head Screw_10-32_2.5in:6 ↔ ELEV_009_BOLTCOVER:2
- Mate:157: ELEV_006_SUPBRK1_THRD:2 ↔ ELEV_009_BOLTCOVER:2
- Mate:158: COTS_90044A121_Black-Oxide Alloy Steel Socket Head Screw_10-32_2.5in:12 ↔ ELEV_009_BOLTCOVER:4
- Mate:159: ELEV_006_SUPBRK1_THRD:1 ↔ ELEV_009_BOLTCOVER:4
- Mate:160: COTS_90044A121_Black-Oxide Alloy Steel Socket Head Screw_10-32_2.5in:10 ↔ ELEV_009_BOLTCOVER:3
- Mate:161: ELEV_006_SUPBRK1_THRD:1 ↔ ELEV_009_BOLTCOVER:3
- Mate:162: COTS_91251A359_Black-Oxide Alloy Steel Socket Head Screw_10-32_2_3-4in:4 ↔ ELEV_010_BOLTCOVER2:1
- Mate:163: COTS_91251A359_Black-Oxide Alloy Steel Socket Head Screw_10-32_2_3-4in:2 ↔ ELEV_010_BOLTCOVER2:2
- Mate:164: COTS_90631A411_Low-Strength Steel Nylon-Insert Locknut_10-32:4 ↔ ELEV_010_BOLTCOVER2:2
- Mate:165: COTS_90631A411_Low-Strength Steel Nylon-Insert Locknut_10-32:3 ↔ ELEV_010_BOLTCOVER2:1
- Mate:166: COTS_91251A359_Black-Oxide Alloy Steel Socket Head Screw_10-32_2_3-4in:3 ↔ ELEV_010_BOLTCOVER2:4
- Mate:167: COTS_91251A359_Black-Oxide Alloy Steel Socket Head Screw_10-32_2_3-4in:1 ↔ ELEV_010_BOLTCOVER2:3
- Mate:168: COTS_90631A411_Low-Strength Steel Nylon-Insert Locknut_10-32:2 ↔ ELEV_010_BOLTCOVER2:4
- Mate:169: COTS_90631A411_Low-Strength Steel Nylon-Insert Locknut_10-32:1 ↔ ELEV_010_BOLTCOVER2:3
- Mate:170: COTS_91251A359_Black-Oxide Alloy Steel Socket Head Screw_10-32_2_3-4in:13 ↔ ELEV_010_BOLTCOVER2:16
- Mate:171: COTS_91251A359_Black-Oxide Alloy Steel Socket Head Screw_10-32_2_3-4in:14 ↔ ELEV_010_BOLTCOVER2:15
- Mate:172: COTS_90631A411_Low-Strength Steel Nylon-Insert Locknut_10-32:14 ↔ ELEV_010_BOLTCOVER2:15
- Mate:173: COTS_90631A411_Low-Strength Steel Nylon-Insert Locknut_10-32:15 ↔ ELEV_010_BOLTCOVER2:16
- Mate:174: COTS_91251A359_Black-Oxide Alloy Steel Socket Head Screw_10-32_2_3-4in:15 ↔ ELEV_010_BOLTCOVER2:14
- Mate:175: COTS_90631A411_Low-Strength Steel Nylon-Insert Locknut_10-32:13 ↔ ELEV_010_BOLTCOVER2:14
- Mate:176: COTS_91251A359_Black-Oxide Alloy Steel Socket Head Screw_10-32_2_3-4in:16 ↔ ELEV_010_BOLTCOVER2:13
- Mate:177: COTS_90631A411_Low-Strength Steel Nylon-Insert Locknut_10-32:16 ↔ ELEV_010_BOLTCOVER2:13
- Mate:178: ELEV_001_BAR1(27.500 in):2 ↔ ELEV_011_EXTRUENDCAP:2
- Mate:180: ELEV_001_BAR1(27.500 in):2 ↔ ELEV_011_EXTRUENDCAP:2
- Mate:181: ELEV_001_BAR1(27.500 in):1 ↔ ELEV_011_EXTRUENDCAP:4
- Mate:182: ELEV_001_BAR1(27.500 in):2 ↔ ELEV_011_EXTRUENDCAP:2
- Mate:183: ELEV_001_BAR1(27.500 in):1 ↔ ELEV_011_EXTRUENDCAP:4
- Mate:184: ELEV_001_BAR1(27.500 in):1 ↔ ELEV_011_EXTRUENDCAP:4
- Mate:186: ELEV_003_BAR3(25.000 in):1 ↔ ELEV_011_EXTRUENDCAP:3
- Mate:187: ELEV_003_BAR3(25.000 in):1 ↔ ELEV_011_EXTRUENDCAP:3
- Mate:188: ELEV_003_BAR3(25.000 in):1 ↔ ELEV_011_EXTRUENDCAP:3
- Mate:189: ELEV_003_BAR3(25.000 in):2 ↔ ELEV_011_EXTRUENDCAP:1
- Mate:190: ELEV_003_BAR3(25.000 in):2 ↔ ELEV_011_EXTRUENDCAP:1
- Mate:191: ELEV_003_BAR3(25.000 in):2 ↔ ELEV_011_EXTRUENDCAP:1
- Mate:192: ELEV_003_BAR3(25.000 in):2 ↔ ELEV_011_EXTRUENDCAP:7
- Mate:193: ELEV_003_BAR3(25.000 in):2 ↔ ELEV_011_EXTRUENDCAP:7
- Mate:194: ELEV_003_BAR3(25.000 in):2 ↔ ELEV_011_EXTRUENDCAP:7
- Mate:195: ELEV_003_BAR3(25.000 in):1 ↔ ELEV_011_EXTRUENDCAP:8
- Mate:196: ELEV_003_BAR3(25.000 in):1 ↔ ELEV_011_EXTRUENDCAP:8
- Mate:197: ELEV_003_BAR3(25.000 in):1 ↔ ELEV_011_EXTRUENDCAP:8
- Mate:198: ELEV_001_BAR1(27.500 in):2 ↔ ELEV_011_EXTRUENDCAP:5
- Mate:199: ELEV_001_BAR1(27.500 in):2 ↔ ELEV_011_EXTRUENDCAP:5
- Mate:200: ELEV_001_BAR1(27.500 in):2 ↔ ELEV_011_EXTRUENDCAP:5
- Mate:201: ELEV_001_BAR1(27.500 in):1 ↔ ELEV_011_EXTRUENDCAP:6
- Mate:202: ELEV_001_BAR1(27.500 in):1 ↔ ELEV_011_EXTRUENDCAP:6
- Mate:203: ELEV_001_BAR1(27.500 in):1 ↔ ELEV_011_EXTRUENDCAP:6
## Named parameters: sa_0 = 35585.8
note: some values were not read from the file. Shown as the stored number, unit unknown: "sa_0".
